# Autodesk Inventor assembly: Base
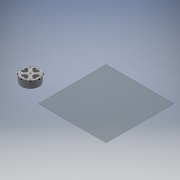
[picture p0: Inventor's stored thumbnail of the model, 180x180]
Saved by Autodesk Inventor 2019 (Build 230136000, 136)
## iProperties
Created: 2020-03-19
Part Number: Base
Document SubType Name: Assembly
Designer: james
Author: james
## Documents named in this file (6)
- F:\JimsRobot\FIRSTRobots\Design\RBX1-REMIX\Base.iam
- F:\JimsRobot\FIRSTRobots\Design\RBX1-REMIX\Table.ipt
- F:\JimsRobot\FIRSTRobots\Design\RBX1-REMIX\base\base_qty1.ipt
- F:\JimsRobot\FIRSTRobots\Design\Library\McMaster\Bearings\5972K910_BALL BEARING 8x22x7.ipt
- F:\JimsRobot\FIRSTRobots\Design\Library\McMaster\Bearings\6153K150_STAINLESS STEEL BALL BEARING 5x16x5.ipt
- F:\JimsRobot\FIRSTRobots\Design\Library\McMaster\SocketScrews\M5-20 91290A242_BLACK-OXIDE CLASS 12.9 SOCKET HEAD CAP SCREW.ipt
## Components (20 placed, 5 different names)
1. Table:1 — Mate:1
2. base_qty1:1 — Mate:1, Mate:2, Mate:3, Mate:4, Mate:5, Mate:6, Mate:7, Mate:8, Mate:9, Mate:10, Mate:11, Mate:12, Mate:13, Mate:14, Mate:15, Mate:16, Mate:17, Mate:18, Mate:19, Mate:20, Mate:21
3. 5972K910_BALL BEARING 8x22x7:1 — Mate:2, Mate:3
4. 5972K910_BALL BEARING 8x22x7:2 — Mate:4, Mate:5
5. 6153K150_STAINLESS STEEL BALL BEARING 5x16x5:1 — Mate:6, Mate:7, Mate:28, Mate:29
6. 6153K150_STAINLESS STEEL BALL BEARING 5x16x5:2 — Mate:8, Mate:9, Mate:26, Mate:27
7. 6153K150_STAINLESS STEEL BALL BEARING 5x16x5:3 — Mate:12, Mate:13, Mate:24, Mate:25
8. 6153K150_STAINLESS STEEL BALL BEARING 5x16x5:4 — Mate:10, Mate:11, Mate:22, Mate:23
9. 6153K150_STAINLESS STEEL BALL BEARING 5x16x5:5 — Mate:14, Mate:15, Mate:36, Mate:37
10. 6153K150_STAINLESS STEEL BALL BEARING 5x16x5:6 — Mate:16, Mate:17, Mate:34, Mate:35
11. 6153K150_STAINLESS STEEL BALL BEARING 5x16x5:7 — Mate:18, Mate:19, Mate:32, Mate:33
12. 6153K150_STAINLESS STEEL BALL BEARING 5x16x5:8 — Mate:20, Mate:21, Mate:30, Mate:31
13. M5-20 91290A242_BLACK-OXIDE CLASS 12.9 SOCKET HEAD CAP SCREW:1 — Mate:26, Mate:27
14. M5-20 91290A242_BLACK-OXIDE CLASS 12.9 SOCKET HEAD CAP SCREW:2 — Mate:24, Mate:25
15. M5-20 91290A242_BLACK-OXIDE CLASS 12.9 SOCKET HEAD CAP SCREW:3 — Mate:28, Mate:29
16. M5-20 91290A242_BLACK-OXIDE CLASS 12.9 SOCKET HEAD CAP SCREW:4 — Mate:30, Mate:31
17. M5-20 91290A242_BLACK-OXIDE CLASS 12.9 SOCKET HEAD CAP SCREW:5 — Mate:32, Mate:33
18. M5-20 91290A242_BLACK-OXIDE CLASS 12.9 SOCKET HEAD CAP SCREW:6 — Mate:36, Mate:37
19. M5-20 91290A242_BLACK-OXIDE CLASS 12.9 SOCKET HEAD CAP SCREW:7 — Mate:34, Mate:35
20. M5-20 91290A242_BLACK-OXIDE CLASS 12.9 SOCKET HEAD CAP SCREW:8 — Mate:22, Mate:23
## Relationships (37: Mate 37)
- Mate:1: Table:1 ↔ base_qty1:1
- Mate:2: base_qty1:1 ↔ 5972K910_BALL BEARING 8x22x7:1
- Mate:3: base_qty1:1 ↔ 5972K910_BALL BEARING 8x22x7:1
- Mate:4: base_qty1:1 ↔ 5972K910_BALL BEARING 8x22x7:2
- Mate:5: base_qty1:1 ↔ 5972K910_BALL BEARING 8x22x7:2
- Mate:6: base_qty1:1 ↔ 6153K150_STAINLESS STEEL BALL BEARING 5x16x5:1
- Mate:7: base_qty1:1 ↔ 6153K150_STAINLESS STEEL BALL BEARING 5x16x5:1
- Mate:8: base_qty1:1 ↔ 6153K150_STAINLESS STEEL BALL BEARING 5x16x5:2
- Mate:9: base_qty1:1 ↔ 6153K150_STAINLESS STEEL BALL BEARING 5x16x5:2
- Mate:10: base_qty1:1 ↔ 6153K150_STAINLESS STEEL BALL BEARING 5x16x5:4
- Mate:11: base_qty1:1 ↔ 6153K150_STAINLESS STEEL BALL BEARING 5x16x5:4
- Mate:12: base_qty1:1 ↔ 6153K150_STAINLESS STEEL BALL BEARING 5x16x5:3
- Mate:13: base_qty1:1 ↔ 6153K150_STAINLESS STEEL BALL BEARING 5x16x5:3
- Mate:14: base_qty1:1 ↔ 6153K150_STAINLESS STEEL BALL BEARING 5x16x5:5
- Mate:15: base_qty1:1 ↔ 6153K150_STAINLESS STEEL BALL BEARING 5x16x5:5
- Mate:16: base_qty1:1 ↔ 6153K150_STAINLESS STEEL BALL BEARING 5x16x5:6
- Mate:17: base_qty1:1 ↔ 6153K150_STAINLESS STEEL BALL BEARING 5x16x5:6
- Mate:18: base_qty1:1 ↔ 6153K150_STAINLESS STEEL BALL BEARING 5x16x5:7
- Mate:19: base_qty1:1 ↔ 6153K150_STAINLESS STEEL BALL BEARING 5x16x5:7
- Mate:20: base_qty1:1 ↔ 6153K150_STAINLESS STEEL BALL BEARING 5x16x5:8
- Mate:21: base_qty1:1 ↔ 6153K150_STAINLESS STEEL BALL BEARING 5x16x5:8
- Mate:22: 6153K150_STAINLESS STEEL BALL BEARING 5x16x5:4 ↔ M5-20 91290A242_BLACK-OXIDE CLASS 12.9 SOCKET HEAD CAP SCREW:8
- Mate:23: 6153K150_STAINLESS STEEL BALL BEARING 5x16x5:4 ↔ M5-20 91290A242_BLACK-OXIDE CLASS 12.9 SOCKET HEAD CAP SCREW:8
- Mate:24: 6153K150_STAINLESS STEEL BALL BEARING 5x16x5:3 ↔ M5-20 91290A242_BLACK-OXIDE CLASS 12.9 SOCKET HEAD CAP SCREW:2
- Mate:25: 6153K150_STAINLESS STEEL BALL BEARING 5x16x5:3 ↔ M5-20 91290A242_BLACK-OXIDE CLASS 12.9 SOCKET HEAD CAP SCREW:2
- Mate:26: 6153K150_STAINLESS STEEL BALL BEARING 5x16x5:2 ↔ M5-20 91290A242_BLACK-OXIDE CLASS 12.9 SOCKET HEAD CAP SCREW:1
- Mate:27: 6153K150_STAINLESS STEEL BALL BEARING 5x16x5:2 ↔ M5-20 91290A242_BLACK-OXIDE CLASS 12.9 SOCKET HEAD CAP SCREW:1
- Mate:28: 6153K150_STAINLESS STEEL BALL BEARING 5x16x5:1 ↔ M5-20 91290A242_BLACK-OXIDE CLASS 12.9 SOCKET HEAD CAP SCREW:3
- Mate:29: 6153K150_STAINLESS STEEL BALL BEARING 5x16x5:1 ↔ M5-20 91290A242_BLACK-OXIDE CLASS 12.9 SOCKET HEAD CAP SCREW:3
- Mate:30: 6153K150_STAINLESS STEEL BALL BEARING 5x16x5:8 ↔ M5-20 91290A242_BLACK-OXIDE CLASS 12.9 SOCKET HEAD CAP SCREW:4
- Mate:31: 6153K150_STAINLESS STEEL BALL BEARING 5x16x5:8 ↔ M5-20 91290A242_BLACK-OXIDE CLASS 12.9 SOCKET HEAD CAP SCREW:4
- Mate:32: 6153K150_STAINLESS STEEL BALL BEARING 5x16x5:7 ↔ M5-20 91290A242_BLACK-OXIDE CLASS 12.9 SOCKET HEAD CAP SCREW:5
- Mate:33: 6153K150_STAINLESS STEEL BALL BEARING 5x16x5:7 ↔ M5-20 91290A242_BLACK-OXIDE CLASS 12.9 SOCKET HEAD CAP SCREW:5
- Mate:34: 6153K150_STAINLESS STEEL BALL BEARING 5x16x5:6 ↔ M5-20 91290A242_BLACK-OXIDE CLASS 12.9 SOCKET HEAD CAP SCREW:7
- Mate:35: 6153K150_STAINLESS STEEL BALL BEARING 5x16x5:6 ↔ M5-20 91290A242_BLACK-OXIDE CLASS 12.9 SOCKET HEAD CAP SCREW:7
- Mate:36: 6153K150_STAINLESS STEEL BALL BEARING 5x16x5:5 ↔ M5-20 91290A242_BLACK-OXIDE CLASS 12.9 SOCKET HEAD CAP SCREW:6
- Mate:37: 6153K150_STAINLESS STEEL BALL BEARING 5x16x5:5 ↔ M5-20 91290A242_BLACK-OXIDE CLASS 12.9 SOCKET HEAD CAP SCREW:6
